# Autodesk Inventor assembly: intakeAsm
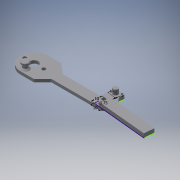
[picture p0: Inventor's stored thumbnail of the model, 180x180]
Saved by Autodesk Inventor 2018.2 (Build 222227000, 227)
## iProperties
Created: 2018-03-18
Part Number: intakeAsm
Document SubType Name: Assembly
Designer: mzhang
Author: mzhang
## Documents named in this file (3)
- C:\Users\mzhang\3D Objects\intakeAsm.iam
- C:\Users\mzhang\3D Objects\grabber.ipt
- C:\Users\mzhang\3D Objects\garabber2.ipt
## Components (2 placed, 2 different names)
1. grabber:1 — Mate:1, Mate:2
2. garabber2:1 — Mate:1, Mate:2
## Relationships (2: Mate 2)
- Mate:1: grabber:1 ↔ garabber2:1
- Mate:2: grabber:1 ↔ garabber2:1
